# Autodesk Inventor assembly: ElectricalHousing2
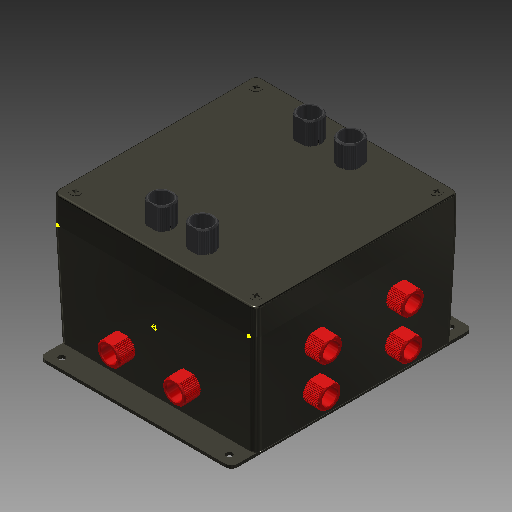
[picture p0: Inventor's stored thumbnail of the model, 512x512]
Saved by Autodesk Inventor 2018 (Build 220112000, 112)
## iProperties
Created: 2019-03-20
Part Number: ElectricalHousing2
Document SubType Name: Assembly
Designer: anirudh
Mass: 530.598 g
Surface Area: 3559.96 cm^2
Volume: 530.598 cm^3
Density: 1 g/cm^3
Author: anirudh
## Documents named in this file (5)
- C:\Users\anirudh\Documents\MARS Fund\MATE Robotics\Silicon Sharks\2018-2019\ElectronicsHousing\Prototype2\ElectricalHousing2.iam
- C:\Users\anirudh\Documents\MARS Fund\MATE Robotics\Silicon Sharks\2018-2019\ElectronicsHousing\Prototype2\AluminumHousing(Master)(2).ipt
- C:\Users\anirudh\Documents\MARS Fund\MATE Robotics\Silicon Sharks\2018-2019\ElectronicsHousing\Prototype2\6MMPenetrator(2).ipt
- C:\Users\anirudh\Documents\MARS Fund\MATE Robotics\Silicon Sharks\2018-2019\ElectronicsHousing\Prototype2\6mmPenetratorORing(2).ipt
- C:\Users\anirudh\Documents\MARS Fund\MATE Robotics\Silicon Sharks\2018-2019\ElectronicsHousing\Prototype2\8MMPenetrator(2).ipt
## Components (33 placed, 4 different names)
1. AluminumHousing(Master)(2):1 — Mate:9, Mate:10, Mate:11, Mate:12, Mate:13, Mate:14, Mate:15, Mate:16, Mate:25, Mate:26, Mate:27, Mate:28, Mate:29, Mate:30, Mate:31, Mate:32, Mate:41, Mate:42, Mate:43, Mate:44, Mate:45, Mate:46, Mate:47, Mate:48, Mate:57, Mate:58, Mate:59, Mate:60, Mate:63, Mate:64, Mate:65, Mate:66
2. 6MMPenetrator(2):1 — Mate:1, Mate:2, Mate:9, Mate:10, Flush:1
3. 6MMPenetrator(2):2 — Mate:3, Mate:4, Mate:11, Mate:12, Flush:1
4. 6MMPenetrator(2):3 — Mate:7, Mate:8, Mate:13, Mate:14, Flush:2
5. 6MMPenetrator(2):4 — Mate:5, Mate:6, Mate:15, Mate:16, Flush:2
6. 6mmPenetratorORing(2):1 — Mate:1, Mate:2
7. 6mmPenetratorORing(2):2 — Mate:3, Mate:4
8. 6mmPenetratorORing(2):3 — Mate:7, Mate:8
9. 6mmPenetratorORing(2):4 — Mate:5, Mate:6
10. 6MMPenetrator(2):5 — Mate:17, Mate:18, Mate:25, Mate:26
11. 6mmPenetratorORing(2):5 — Mate:17, Mate:18
12. 6MMPenetrator(2):6 — Mate:19, Mate:20, Mate:27, Mate:28
13. 6mmPenetratorORing(2):6 — Mate:19, Mate:20
14. 6MMPenetrator(2):7 — Mate:23, Mate:24, Mate:29, Mate:30
15. 6mmPenetratorORing(2):7 — Mate:23, Mate:24
16. 6MMPenetrator(2):8 — Mate:21, Mate:22, Mate:31, Mate:32
17. 6mmPenetratorORing(2):8 — Mate:21, Mate:22
18. 6MMPenetrator(2):9 — Mate:33, Mate:34, Mate:41, Mate:42
19. 6mmPenetratorORing(2):9 — Mate:33, Mate:34
20. 6MMPenetrator(2):10 — Mate:35, Mate:36, Mate:45, Mate:46
21. 6mmPenetratorORing(2):10 — Mate:35, Mate:36
22. 6MMPenetrator(2):11 — Mate:39, Mate:40, Mate:47, Mate:48
23. 6mmPenetratorORing(2):11 — Mate:39, Mate:40
24. 6MMPenetrator(2):12 — Mate:37, Mate:38, Mate:43, Mate:44
25. 6mmPenetratorORing(2):12 — Mate:37, Mate:38
26. 6mmPenetratorORing(2):13 — Mate:61, Mate:62
27. 8MMPenetrator(2):1 — Mate:61, Mate:62, Mate:63, Mate:64
28. 6mmPenetratorORing(2):14 — Mate:55, Mate:56
29. 8MMPenetrator(2):2 — Mate:55, Mate:56, Mate:65, Mate:66
30. 6mmPenetratorORing(2):15 — Mate:51, Mate:52
31. 8MMPenetrator(2):3 — Mate:51, Mate:52, Mate:59, Mate:60
32. 6mmPenetratorORing(2):16 — Mate:49, Mate:50
33. 8MMPenetrator(2):4 — Mate:49, Mate:50, Mate:57, Mate:58
## Relationships (66: Mate 64, Flush 2)
- Mate:1: 6MMPenetrator(2):1 ↔ 6mmPenetratorORing(2):1
- Mate:2: 6MMPenetrator(2):1 ↔ 6mmPenetratorORing(2):1
- Mate:3: 6MMPenetrator(2):2 ↔ 6mmPenetratorORing(2):2
- Mate:4: 6MMPenetrator(2):2 ↔ 6mmPenetratorORing(2):2
- Mate:5: 6MMPenetrator(2):4 ↔ 6mmPenetratorORing(2):4
- Mate:6: 6MMPenetrator(2):4 ↔ 6mmPenetratorORing(2):4
- Mate:7: 6MMPenetrator(2):3 ↔ 6mmPenetratorORing(2):3
- Mate:8: 6MMPenetrator(2):3 ↔ 6mmPenetratorORing(2):3
- Mate:9: AluminumHousing(Master)(2):1 ↔ 6MMPenetrator(2):1
- Mate:10: AluminumHousing(Master)(2):1 ↔ 6MMPenetrator(2):1
- Mate:11: AluminumHousing(Master)(2):1 ↔ 6MMPenetrator(2):2
- Mate:12: AluminumHousing(Master)(2):1 ↔ 6MMPenetrator(2):2
- Flush:1: 6MMPenetrator(2):1 ↔ 6MMPenetrator(2):2
- Mate:13: AluminumHousing(Master)(2):1 ↔ 6MMPenetrator(2):3
- Mate:14: AluminumHousing(Master)(2):1 ↔ 6MMPenetrator(2):3
- Mate:15: AluminumHousing(Master)(2):1 ↔ 6MMPenetrator(2):4
- Mate:16: AluminumHousing(Master)(2):1 ↔ 6MMPenetrator(2):4
- Flush:2: 6MMPenetrator(2):3 ↔ 6MMPenetrator(2):4
- Mate:17: 6MMPenetrator(2):5 ↔ 6mmPenetratorORing(2):5
- Mate:18: 6MMPenetrator(2):5 ↔ 6mmPenetratorORing(2):5
- Mate:19: 6MMPenetrator(2):6 ↔ 6mmPenetratorORing(2):6
- Mate:20: 6MMPenetrator(2):6 ↔ 6mmPenetratorORing(2):6
- Mate:21: 6MMPenetrator(2):8 ↔ 6mmPenetratorORing(2):8
- Mate:22: 6MMPenetrator(2):8 ↔ 6mmPenetratorORing(2):8
- Mate:23: 6MMPenetrator(2):7 ↔ 6mmPenetratorORing(2):7
- Mate:24: 6MMPenetrator(2):7 ↔ 6mmPenetratorORing(2):7
- Mate:25: AluminumHousing(Master)(2):1 ↔ 6MMPenetrator(2):5
- Mate:26: AluminumHousing(Master)(2):1 ↔ 6MMPenetrator(2):5
- Mate:27: AluminumHousing(Master)(2):1 ↔ 6MMPenetrator(2):6
- Mate:28: AluminumHousing(Master)(2):1 ↔ 6MMPenetrator(2):6
- Mate:29: AluminumHousing(Master)(2):1 ↔ 6MMPenetrator(2):7
- Mate:30: AluminumHousing(Master)(2):1 ↔ 6MMPenetrator(2):7
- Mate:31: AluminumHousing(Master)(2):1 ↔ 6MMPenetrator(2):8
- Mate:32: AluminumHousing(Master)(2):1 ↔ 6MMPenetrator(2):8
- Mate:33: 6MMPenetrator(2):9 ↔ 6mmPenetratorORing(2):9
- Mate:34: 6MMPenetrator(2):9 ↔ 6mmPenetratorORing(2):9
- Mate:35: 6MMPenetrator(2):10 ↔ 6mmPenetratorORing(2):10
- Mate:36: 6MMPenetrator(2):10 ↔ 6mmPenetratorORing(2):10
- Mate:37: 6MMPenetrator(2):12 ↔ 6mmPenetratorORing(2):12
- Mate:38: 6MMPenetrator(2):12 ↔ 6mmPenetratorORing(2):12
- Mate:39: 6MMPenetrator(2):11 ↔ 6mmPenetratorORing(2):11
- Mate:40: 6MMPenetrator(2):11 ↔ 6mmPenetratorORing(2):11
- Mate:41: AluminumHousing(Master)(2):1 ↔ 6MMPenetrator(2):9
- Mate:42: AluminumHousing(Master)(2):1 ↔ 6MMPenetrator(2):9
- Mate:43: AluminumHousing(Master)(2):1 ↔ 6MMPenetrator(2):12
- Mate:44: AluminumHousing(Master)(2):1 ↔ 6MMPenetrator(2):12
- Mate:45: AluminumHousing(Master)(2):1 ↔ 6MMPenetrator(2):10
- Mate:46: AluminumHousing(Master)(2):1 ↔ 6MMPenetrator(2):10
- Mate:47: AluminumHousing(Master)(2):1 ↔ 6MMPenetrator(2):11
- Mate:48: AluminumHousing(Master)(2):1 ↔ 6MMPenetrator(2):11
- Mate:49: 6mmPenetratorORing(2):16 ↔ 8MMPenetrator(2):4
- Mate:50: 6mmPenetratorORing(2):16 ↔ 8MMPenetrator(2):4
- Mate:51: 6mmPenetratorORing(2):15 ↔ 8MMPenetrator(2):3
- Mate:52: 6mmPenetratorORing(2):15 ↔ 8MMPenetrator(2):3
- Mate:55: 6mmPenetratorORing(2):14 ↔ 8MMPenetrator(2):2
- Mate:56: 6mmPenetratorORing(2):14 ↔ 8MMPenetrator(2):2
- Mate:57: AluminumHousing(Master)(2):1 ↔ 8MMPenetrator(2):4
- Mate:58: AluminumHousing(Master)(2):1 ↔ 8MMPenetrator(2):4
- Mate:59: AluminumHousing(Master)(2):1 ↔ 8MMPenetrator(2):3
- Mate:60: AluminumHousing(Master)(2):1 ↔ 8MMPenetrator(2):3
- Mate:61: 6mmPenetratorORing(2):13 ↔ 8MMPenetrator(2):1
- Mate:62: 6mmPenetratorORing(2):13 ↔ 8MMPenetrator(2):1
- Mate:63: AluminumHousing(Master)(2):1 ↔ 8MMPenetrator(2):1
- Mate:64: AluminumHousing(Master)(2):1 ↔ 8MMPenetrator(2):1
- Mate:65: AluminumHousing(Master)(2):1 ↔ 8MMPenetrator(2):2
- Mate:66: AluminumHousing(Master)(2):1 ↔ 8MMPenetrator(2):2
